# Autodesk Inventor assembly: hashikadai1
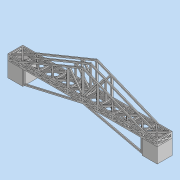
[picture p0: Inventor's stored thumbnail of the model, 180x180]
Saved by Autodesk Inventor 2022 (Build 260153000, 153)
## iProperties
Created: 2024-05-14
Part Number: hashikadai1
Document SubType Name: Assembly
Designer: ktamu
Mass: 403.339 g
Surface Area: 1722.35 cm^2
Volume: 403.339 cm^3
Density: 1 g/cm^3
Author: ktamu
## Documents named in this file (10)
- D:\SDinventor\DesignHashi\DesignHashi9-1c-7-3M1widelowDouble - コピー\hashikadai1.iam
- D:\SDinventor\DesignHashi\DesignHashi9-1c-7-3M1widelowDouble - コピー\hashgeta1.ipt
- D:\SDinventor\DesignHashi\DesignHashi9-1c-7-3M1widelowDouble - コピー\hashi1shado.ipt
- D:\SDinventor\DesignHashi\DesignHashi9-1c-7-3M1widelowDouble - コピー\loadstick.ipt
- D:\SDinventor\DesignHashi\DesignHashi9-1c-7-3M1widelowDouble - コピー\hashikadai1\AIP\FEA\ep6vs5l7k.ftes
- D:\SDinventor\DesignHashi\DesignHashi9-1c-7-3M1widelowDouble - コピー\hashikadai1\AIP\FEA\ep6vs5l7k.fwiz
- D:\SDinventor\DesignHashi\DesignHashi9-1c-7-3M1widelowDouble - コピー\hashikadai1\AIP\FEA\ep6vs5l9c.fmsh
- D:\SDinventor\DesignHashi\DesignHashi9-1c-7-3M1widelowDouble - コピー\hashikadai1\AIP\FEA\ep6vs5l9d.fres
- D:\SDinventor\DesignHashi\DesignHashi9-1c-7-3M1widelowDouble - コピー\hashikadai1\AIP\FEA\ep6vs5l7k.fins
- D:\SDinventor\DesignHashi\DesignHashi9-1c-7-3M1widelowDouble - コピー\hashikadai1\AIP\FEA\ep6vs5l7k.fsat
## Components (4 placed, 3 different names)
1. hashgeta1:1 — フラッシュ:2, フラッシュ:3
2. hashi1shado:1 — フラッシュ:1, フラッシュ:2, フラッシュ:3, フラッシュ:4, メイト:1, フラッシュ:5, フラッシュ:6
3. hashgeta1:2 — フラッシュ:1, フラッシュ:4
4. loadstick:1 — メイト:1, フラッシュ:5, フラッシュ:6
## Relationships (7: Flush 6, Mate 1)
- フラッシュ:1 [Flush]: hashi1shado:1 ↔ hashgeta1:2
- フラッシュ:2 [Flush]: hashgeta1:1 ↔ hashi1shado:1
- フラッシュ:3 [Flush]: hashgeta1:1 ↔ hashi1shado:1
- フラッシュ:4 [Flush]: hashi1shado:1 ↔ hashgeta1:2
- メイト:1 [Mate]: hashi1shado:1 ↔ loadstick:1
- フラッシュ:5 [Flush]: hashi1shado:1 ↔ loadstick:1
- フラッシュ:6 [Flush] (248 mm): hashi1shado:1 ↔ loadstick:1
